# Autodesk Inventor assembly: FullAssembly
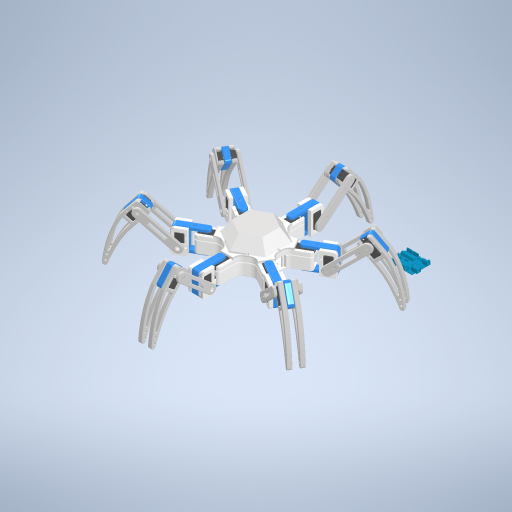
[picture p0: Inventor's stored thumbnail of the model, 512x512]
Saved by Autodesk Inventor 2024 (Build 280153000, 153)
## iProperties
Created: 2026-01-28
Part Number: FullAssembly
Document SubType Name: Assembly
Designer: Liam
Mass: 931.394 g
Surface Area: 3473.48 cm^2
Volume: 931.394 cm^3
Density: 1 g/cm^3
Author: Liam
## Documents named in this file (6)
- C:\Users\Liam\OneDrive\Documents\Inventor\Hexapod\FullAssembly.iam
- C:\Users\Liam\OneDrive\Documents\Inventor\Hexapod\LegAssembly.iam
- C:\Users\Liam\OneDrive\Documents\Inventor\Hexapod\BaseBottomHex.ipt
- C:\Users\Liam\OneDrive\Documents\Inventor\Hexapod\BaseTopHex.ipt
- C:\Users\Liam\OneDrive\Documents\Inventor\Electronics\Arduino-UNO\Arduino-UNO.iam
- C:\Users\Liam\OneDrive\Documents\Inventor\Hexapod\HexPivot.ipt
## Components (10 placed, 5 different names)
1. LegAssembly:1 [sub-assembly] — Rigid:3
2. BaseBottomHex:1 — Rigid:2, Rigid:3, Rigid:4, Rigid:5, Rigid:6, Rigid:7, Rigid:8, Rigid:9
3. Arduino-UNO:1 [sub-assembly]
4. HexPivot:1 — Rigid:2
5. BaseTopHex:1 — Rigid:4
6. LegAssembly:2 [sub-assembly] — Rigid:5
7. LegAssembly:3 [sub-assembly] — Rigid:6
8. LegAssembly:4 [sub-assembly] — Rigid:7
9. LegAssembly:5 [sub-assembly] — Rigid:8
10. LegAssembly:6 [sub-assembly] — Rigid:9
## Relationships (8: WeldJoint 8)
- Rigid:2 [WeldJoint]: BaseBottomHex:1 ↔ HexPivot:1
- Rigid:3 [WeldJoint]: LegAssembly:1 ↔ BaseBottomHex:1
- Rigid:4 [WeldJoint]: BaseBottomHex:1 ↔ BaseTopHex:1
- Rigid:5 [WeldJoint]: BaseBottomHex:1 ↔ LegAssembly:2
- Rigid:6 [WeldJoint]: BaseBottomHex:1 ↔ LegAssembly:3
- Rigid:7 [WeldJoint]: BaseBottomHex:1 ↔ LegAssembly:4
- Rigid:8 [WeldJoint]: BaseBottomHex:1 ↔ LegAssembly:5
- Rigid:9 [WeldJoint]: BaseBottomHex:1 ↔ LegAssembly:6
